# Autodesk Inventor assembly: drivetrain_assembly
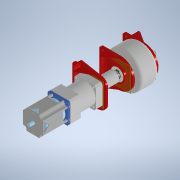
[picture p0: Inventor's stored thumbnail of the model, 180x180]
Saved by Autodesk Inventor 2021.3 (Build 253353000, 353)
## iProperties
Created: 2023-04-09
Part Number: drivetrain_assembly
Document SubType Name: Assembly
Designer: nxf77172
Author: nxf77172
## Documents named in this file (4)
- C:\Users\nxf77172\Desktop\mechanical_cleaned\custom_parts\drivetrain\drivetrain_assembly.iam
- C:\Users\nxf77172\Desktop\mechanical_cleaned\custom_parts\drivetrain\motor assembly.iam
- C:\Users\nxf77172\Desktop\mechanical_cleaned\custom_parts\drivetrain\wheel_assembly.iam
- C:\Users\nxf77172\Desktop\mechanical_cleaned\custom_parts\drivetrain\14mm_shaft_coupler.ipt
## Components (3 placed, 3 different names)
1. motor assembly:1 [sub-assembly] — Angle:1, Flush:1, Flush:2, Mate:1, Mate:2, Mate:3
2. wheel_assembly:1 [sub-assembly] — Angle:1, Flush:1, Flush:2, Mate:1, Mate:4, Angle:2
3. 14mm_shaft_coupler:1 — Mate:2, Mate:3, Mate:4, Angle:2
## Relationships (8: Mate 4, Angle 2, Flush 2)
- Angle:1 (0 deg): motor assembly:1 ↔ wheel_assembly:1
- Flush:1: motor assembly:1 ↔ wheel_assembly:1
- Flush:2 (75 mm): motor assembly:1 ↔ wheel_assembly:1
- Mate:1: motor assembly:1 ↔ wheel_assembly:1
- Mate:2: motor assembly:1 ↔ 14mm_shaft_coupler:1
- Mate:3: motor assembly:1 ↔ 14mm_shaft_coupler:1
- Mate:4 (10 mm): wheel_assembly:1 ↔ 14mm_shaft_coupler:1
- Angle:2 (-90 deg): wheel_assembly:1 ↔ 14mm_shaft_coupler:1
